# Autodesk Inventor assembly: Mohinh3D
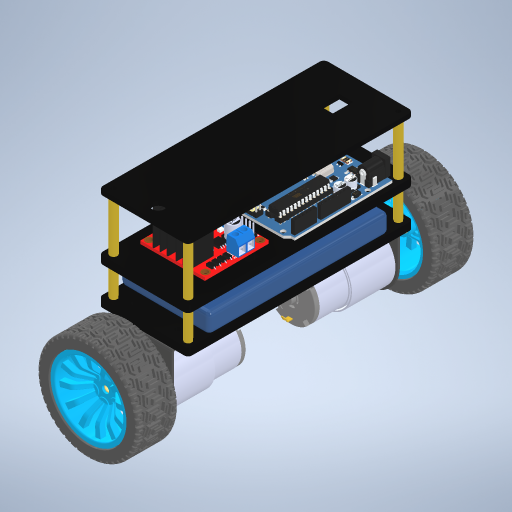
[picture p0: Inventor's stored thumbnail of the model, 512x512]
Saved by Autodesk Inventor 2023 (Build 270158000, 158)
## iProperties
Created: 2015-12-06
Part Number: Mohinh3D
Description: STEP AP214
Document SubType Name: Assembly
Designer: Admins
Sending System: SolidWorks 2014
Preprocessor: SwSTEP 2.0
Title: JGA25-371_ASM_(AP214).STEP
Revision Number: ANY
## Documents named in this file (12)
- D:\UNI\DoAn2\HardwareDesign\Mohinh3D.iam
- D:\UNI\DoAn2\HardwareDesign\65mm-wheel-1.snapshot.1\蓝色轮胎\65mm蓝色轮胎总装-实际外径68mm_MIR.ipt
- D:\UNI\DoAn2\HardwareDesign\l298-module-1.snapshot.14\L298N Stepper Motor Driver (Red)_MIR.ipt
- D:\UNI\DoAn2\HardwareDesign\arduino-uno-r3-8.snapshot.2\Arduino Uno_MIR.ipt
- D:\UNI\DoAn2\DeDuoi_MIR.ipt
- D:\UNI\DoAn2\DeGiua_MIR.ipt
- D:\UNI\DoAn2\HardwareDesign\37-mm-dc-geared-motor-mounting-bracket-1.snapshot.11\37 mm DC Geared Motor Mounting Bracket_MIR.ipt
- D:\UNI\DoAn2\HardwareDesign\jgb37-520-1.snapshot.2\JGB37-520_MIR.ipt
- D:\UNI\DoAn2\HardwareDesign\Trudong30_MIR.ipt
- D:\UNI\DoAn2\HardwareDesign\Trudong35_MIR.ipt
- D:\UNI\DoAn2\HardwareDesign\MatTren_MIR.ipt
- D:\UNI\DoAn2\HardwareDesign\Battery.ipt
## Components (20 placed, 11 different names)
1. 65mm蓝色轮胎总装-实际外径68mm_MIR:1 — Mate:82, Mate:83
2. 65mm蓝色轮胎总装-实际外径68mm_MIR:2 — Mate:87, Mate:88
3. L298N Stepper Motor Driver (Red)_MIR:1 — Mate:74, Mate:75
4. Arduino Uno_MIR:1 — Mate:72, Mate:73
5. DeDuoi_MIR:1 — Mate:76, Mate:77, Mate:78, Mate:79, Mate:80, Mate:81, Mate:92, Mate:93, Mate:94, Mate:97, Mate:101, Mate:102, Mate:106, Mate:107, Mate:114, Flush:1
6. DeGiua_MIR:1 — Mate:72, Mate:73, Mate:74, Mate:75, Mate:95, Mate:96, Mate:98, Mate:99, Mate:100, Mate:103, Mate:104, Mate:105, Mate:108, Mate:110
7. 37 mm DC Geared Motor Mounting Bracket_MIR:1 — Mate:76, Mate:77, Mate:78, Mate:84, Mate:85, Mate:86
8. 37 mm DC Geared Motor Mounting Bracket_MIR:2 — Mate:79, Mate:80, Mate:81, Mate:89, Mate:90, Mate:91
9. JGB37-520_MIR:1 — Mate:82, Mate:83, Mate:84, Mate:85, Mate:86
10. JGB37-520_MIR:2 — Mate:87, Mate:88, Mate:89, Mate:90, Mate:91
11. Trudong30_MIR:1 — Mate:92, Mate:93, Mate:94
12. Trudong35_MIR:1 — Mate:95, Mate:96
13. Trudong30_MIR:2 — Mate:97, Mate:98
14. Trudong35_MIR:2 — Mate:99, Mate:100, Mate:113
15. Trudong30_MIR:3 — Mate:101, Mate:102, Mate:103, Mate:109
16. Trudong35_MIR:3 — Mate:104, Mate:105, Mate:115
17. Trudong30_MIR:4 — Mate:106, Mate:107, Mate:115
18. Trudong35_MIR:4 — Mate:108, Mate:109, Mate:110, Mate:111, Mate:112
19. MatTren_MIR:1 — Mate:111, Mate:112, Mate:113
20. Battery:1 — Mate:114, Flush:1
## Relationships (45: Mate 44, Flush 1)
- Mate:72: Arduino Uno_MIR:1 ↔ DeGiua_MIR:1
- Mate:73: Arduino Uno_MIR:1 ↔ DeGiua_MIR:1
- Mate:74: L298N Stepper Motor Driver (Red)_MIR:1 ↔ DeGiua_MIR:1
- Mate:75: L298N Stepper Motor Driver (Red)_MIR:1 ↔ DeGiua_MIR:1
- Mate:76: DeDuoi_MIR:1 ↔ 37 mm DC Geared Motor Mounting Bracket_MIR:1
- Mate:77: DeDuoi_MIR:1 ↔ 37 mm DC Geared Motor Mounting Bracket_MIR:1
- Mate:78: DeDuoi_MIR:1 ↔ 37 mm DC Geared Motor Mounting Bracket_MIR:1
- Mate:79: DeDuoi_MIR:1 ↔ 37 mm DC Geared Motor Mounting Bracket_MIR:2
- Mate:80: DeDuoi_MIR:1 ↔ 37 mm DC Geared Motor Mounting Bracket_MIR:2
- Mate:81: DeDuoi_MIR:1 ↔ 37 mm DC Geared Motor Mounting Bracket_MIR:2
- Mate:82: 65mm蓝色轮胎总装-实际外径68mm_MIR:1 ↔ JGB37-520_MIR:1
- Mate:83: 65mm蓝色轮胎总装-实际外径68mm_MIR:1 ↔ JGB37-520_MIR:1
- Mate:84: 37 mm DC Geared Motor Mounting Bracket_MIR:1 ↔ JGB37-520_MIR:1
- Mate:85: 37 mm DC Geared Motor Mounting Bracket_MIR:1 ↔ JGB37-520_MIR:1
- Mate:86: 37 mm DC Geared Motor Mounting Bracket_MIR:1 ↔ JGB37-520_MIR:1
- Mate:87: 65mm蓝色轮胎总装-实际外径68mm_MIR:2 ↔ JGB37-520_MIR:2
- Mate:88: 65mm蓝色轮胎总装-实际外径68mm_MIR:2 ↔ JGB37-520_MIR:2
- Mate:89: 37 mm DC Geared Motor Mounting Bracket_MIR:2 ↔ JGB37-520_MIR:2
- Mate:90: 37 mm DC Geared Motor Mounting Bracket_MIR:2 ↔ JGB37-520_MIR:2
- Mate:91: 37 mm DC Geared Motor Mounting Bracket_MIR:2 ↔ JGB37-520_MIR:2
- Mate:92: DeDuoi_MIR:1 ↔ Trudong30_MIR:1
- Mate:93: DeDuoi_MIR:1 ↔ Trudong30_MIR:1
- Mate:94: DeDuoi_MIR:1 ↔ Trudong30_MIR:1
- Mate:95: DeGiua_MIR:1 ↔ Trudong35_MIR:1
- Mate:96: DeGiua_MIR:1 ↔ Trudong35_MIR:1
- Mate:97: DeDuoi_MIR:1 ↔ Trudong30_MIR:2
- Mate:98: DeGiua_MIR:1 ↔ Trudong30_MIR:2
- Mate:99: DeGiua_MIR:1 ↔ Trudong35_MIR:2
- Mate:100: DeGiua_MIR:1 ↔ Trudong35_MIR:2
- Mate:101: DeDuoi_MIR:1 ↔ Trudong30_MIR:3
- Mate:102: DeDuoi_MIR:1 ↔ Trudong30_MIR:3
- Mate:103: DeGiua_MIR:1 ↔ Trudong30_MIR:3
- Mate:104: DeGiua_MIR:1 ↔ Trudong35_MIR:3
- Mate:105: DeGiua_MIR:1 ↔ Trudong35_MIR:3
- Mate:106: DeDuoi_MIR:1 ↔ Trudong30_MIR:4
- Mate:107: DeDuoi_MIR:1 ↔ Trudong30_MIR:4
- Mate:108: DeGiua_MIR:1 ↔ Trudong35_MIR:4
- Mate:109: Trudong30_MIR:3 ↔ Trudong35_MIR:4
- Mate:110: DeGiua_MIR:1 ↔ Trudong35_MIR:4
- Mate:111: Trudong35_MIR:4 ↔ MatTren_MIR:1
- Mate:112: Trudong35_MIR:4 ↔ MatTren_MIR:1
- Mate:113: Trudong35_MIR:2 ↔ MatTren_MIR:1
- Mate:114: DeDuoi_MIR:1 ↔ Battery:1
- Flush:1: DeDuoi_MIR:1 ↔ Battery:1
- Mate:115: Trudong35_MIR:3 ↔ Trudong30_MIR:4
